# Autodesk Inventor assembly: assemblage
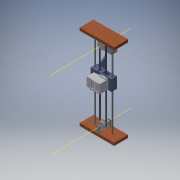
[picture p0: Inventor's stored thumbnail of the model, 180x180]
Saved by Autodesk Inventor 2017 (Build 210142000, 142)
## iProperties
Created: 2017-10-26
Part Number: assemblage
Document SubType Name: Assembly
Designer: Biscuit
Author: Biscuit
## Documents named in this file (11)
- C:\Users\Biscuit\Google Drive\ENSEIRB\EIRBOT\COUPE 2018\Cubes\assemblage.iam
- C:\Users\Biscuit\Google Drive\ENSEIRB\EIRBOT\COUPE 2018\Cubes\extremite.ipt
- C:\Users\Biscuit\Google Drive\ENSEIRB\EIRBOT\COUPE 2018\Cubes\axes.ipt
- C:\Users\Biscuit\Google Drive\ENSEIRB\EIRBOT\COUPE 2018\Cubes\SupportPlateau.ipt
- C:\Users\Biscuit\Google Drive\ENSEIRB\EIRBOT\COUPE 2018\Cubes\supportPoulie.ipt
- C:\Users\Biscuit\Google Drive\ENSEIRB\EIRBOT\COUPE 2018\Cubes\moteur.ipt
- C:\Users\Biscuit\Google Drive\ENSEIRB\EIRBOT\COUPE 2018\Cubes\axe_poulie.ipt
- C:\Users\Biscuit\Google Drive\ENSEIRB\EIRBOT\COUPE 2018\Cubes\assemblage\Design Accelerator\Synchronous Belts Transmission1.iam
- C:\Users\Biscuit\Google Drive\ENSEIRB\EIRBOT\COUPE 2018\Cubes\extremite_pince.ipt
- C:\Users\Biscuit\Google Drive\ENSEIRB\EIRBOT\COUPE 2018\Cubes\assemblage\Design Accelerator\Shaft1.iam
- C:\Users\Biscuit\Google Drive\ENSEIRB\EIRBOT\COUPE 2018\Cubes\ax12.iam
## Components (13 placed, 10 different names)
1. extremite:1 — Mate:3, Mate:4, Mate:5, Mate:6, Flush:1, Mate:11, Mate:12, Mate:13, Mate:14
2. extremite:2 — Mate:7, Mate:8, Mate:9, Mate:15, Flush:6, Flush:7
3. axes:1 — Mate:4, Mate:5, Mate:9, Mate:10, Mate:25
4. axes:2 — Mate:3, Mate:6, Mate:7, Mate:8, Mate:26
5. SupportPlateau:1 — Mate:10, Flush:1, Mate:35, Mate:36, Mate:37, Mate:38, Angle:1, Mate:39, Mate:40, Mate:41
6. supportPoulie:1 — Mate:11, Flush:2, Mate:14, Mate:33
7. supportPoulie:2 — Mate:12, Flush:2, Mate:13, Mate:24, Flush:5
8. moteur:1 — Mate:15, Flush:6, Flush:7, Mate:30, Mate:31
9. axe_poulie:1 — Mate:24, Flush:5, Mate:29
10. Synchronous Belts Transmission:1 [sub-assembly]
11. extremite_pince:1 — Mate:35, Mate:36
12. Shaft:1 [sub-assembly] — Mate:37, Mate:38, Angle:1
13. ax12:1 [sub-assembly] — Mate:39, Mate:40, Mate:41
## Relationships (37: Mate 31, Flush 5, Angle 1)
- Mate:3: extremite:1 ↔ axes:2
- Mate:4: extremite:1 ↔ axes:1
- Mate:5: extremite:1 ↔ axes:1
- Mate:6: extremite:1 ↔ axes:2
- Mate:7: extremite:2 ↔ axes:2
- Mate:8: extremite:2 ↔ axes:2
- Mate:9: extremite:2 ↔ axes:1
- Mate:10: axes:1 ↔ SupportPlateau:1
- Flush:1: extremite:1 ↔ SupportPlateau:1
- Mate:11: extremite:1 ↔ supportPoulie:1
- Mate:12: extremite:1 ↔ supportPoulie:2
- Flush:2: supportPoulie:1 ↔ supportPoulie:2
- Mate:13: extremite:1 ↔ supportPoulie:2
- Mate:14: extremite:1 ↔ supportPoulie:1
- Mate:15: extremite:2 ↔ moteur:1
- Mate:24: supportPoulie:2 ↔ axe_poulie:1
- Flush:5: supportPoulie:2 ↔ axe_poulie:1
- Mate:25: axes:1
- Mate:26: axes:2
- Mate:27
- Mate:28
- Flush:6 (39 mm): extremite:2 ↔ moteur:1
- Flush:7: extremite:2 ↔ moteur:1
- Mate:29: axe_poulie:1
- Mate:30: moteur:1
- Mate:31: moteur:1
- Mate:32
- Mate:33: supportPoulie:1
- Mate:34
- Mate:35: SupportPlateau:1 ↔ extremite_pince:1
- Mate:36: SupportPlateau:1 ↔ extremite_pince:1
- Mate:37: SupportPlateau:1 ↔ Shaft:1
- Mate:38: SupportPlateau:1 ↔ Shaft:1
- Angle:1 (0 deg): SupportPlateau:1 ↔ Shaft:1
- Mate:39: SupportPlateau:1 ↔ ax12:1
- Mate:40: SupportPlateau:1 ↔ ax12:1
- Mate:41: SupportPlateau:1 ↔ ax12:1
